# Autodesk Inventor assembly: einzel_assembly
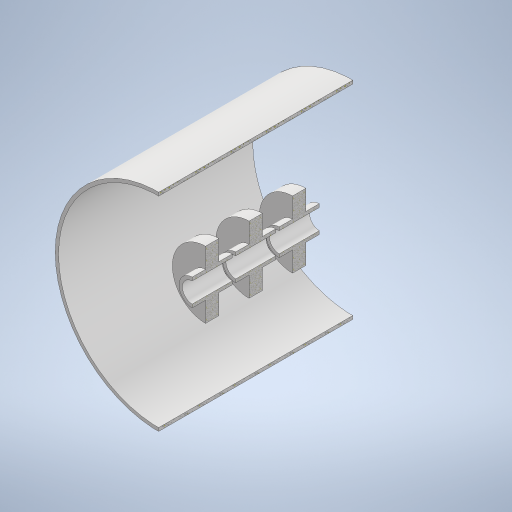
[picture p0: Inventor's stored thumbnail of the model, 512x512]
Saved by Autodesk Inventor 2024 (Build 280153000, 153)
## iProperties
Created: 2023-11-17
Part Number: einzel_assembly
Document SubType Name: Assembly
Designer: h2p_l
Author: h2p_l
## Documents named in this file (3)
- C:\Users\h2p_l\Desktop\ion_trajectory_integrator\MISC_happy_hour_example\einzel_assembly.iam
- C:\Users\h2p_l\Desktop\ion_trajectory_integrator\MISC_happy_hour_example\einzel_element.ipt
- C:\Users\h2p_l\Desktop\ion_trajectory_integrator\MISC_happy_hour_example\shield.ipt
## Components (4 placed, 2 different names)
1. einzel_element:1 — Mate:1, Mate:2, Mate:6
2. einzel_element:2 — Mate:1, Mate:2, Mate:3, Mate:4, Mate:5
3. einzel_element:3 — Mate:3, Mate:4
4. shield:1 — Mate:5, Mate:6
## Relationships (6: Mate 6)
- Mate:1 (0.5 mm): einzel_element:1 ↔ einzel_element:2
- Mate:2: einzel_element:1 ↔ einzel_element:2
- Mate:3 (0.5 mm): einzel_element:2 ↔ einzel_element:3
- Mate:4: einzel_element:2 ↔ einzel_element:3
- Mate:5: einzel_element:2 ↔ shield:1
- Mate:6 (-5 mm): einzel_element:1 ↔ shield:1
